# Autodesk Inventor assembly: V_156_1C25
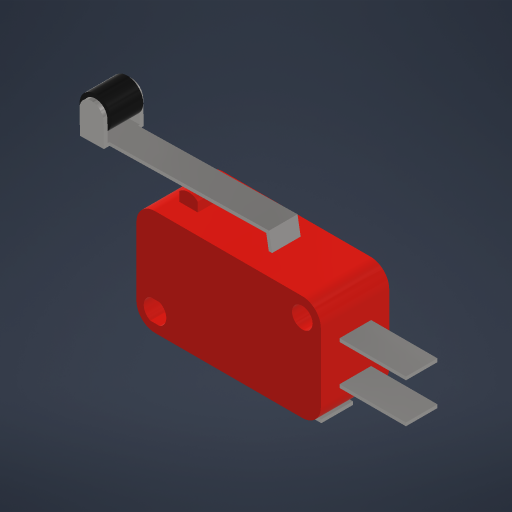
[picture p0: Inventor's stored thumbnail of the model, 512x512]
Saved by Autodesk Inventor 2024.1 (Build 281209000, 209)
## iProperties
Created: 2011-02-19
Part Number: V_156_1C25
Description: STEP AP203
Document SubType Name: Assembly
Designer: jaege
Sending System: SolidWorks 2002025
Preprocessor: SwSTEP 2.0
Title: V_156_1C25.step
Author: OSMC1.0
Revision Number: ANY
## Documents named in this file (3)
- C:\Users\jaege\VUB\Schakel_Ind_Elo\Year_1_Both\BA_Thesis\3D_Files\Lift_V2\LimitSwitch_Big.iam
- C:\Users\jaege\VUB\Schakel_Ind_Elo\Year_1_Both\BA_Thesis\3D_Files\Lift_V2\V_156_1C25_STEP\V_156_1C25\V_156_1C25_BASE.ipt
- C:\Users\jaege\VUB\Schakel_Ind_Elo\Year_1_Both\BA_Thesis\3D_Files\Lift_V2\V_156_1C25_STEP\V_156_1C25\V_156_1C25_ACTUATOR.ipt
## Components (2 placed, 2 different names)
1. V_156_1C25_BASE_1 — Mate:1, Mate:2, Flush:1, Mate:3
2. V_156_1C25_ACTUATOR_2 — Mate:1, Mate:2, Flush:1, Mate:3
## Relationships (4: Mate 3, Flush 1)
- Mate:1: V_156_1C25_BASE_1 ↔ V_156_1C25_ACTUATOR_2
- Mate:2 (7.9 mm): V_156_1C25_BASE_1 ↔ V_156_1C25_ACTUATOR_2
- Flush:1 (2.6467 mm): V_156_1C25_BASE_1 ↔ V_156_1C25_ACTUATOR_2
- Mate:3 (3.8418 mm): V_156_1C25_BASE_1 ↔ V_156_1C25_ACTUATOR_2
